# Autodesk Inventor assembly: ferris_wheel_assy1
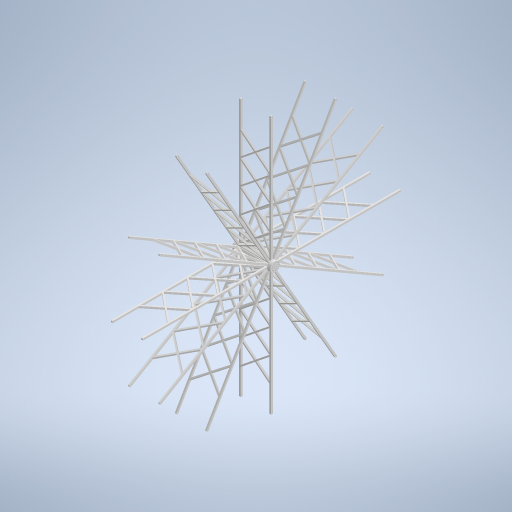
[picture p0: Inventor's stored thumbnail of the model, 512x512]
Saved by Autodesk Inventor 2023 (Build 270158000, 158)
## iProperties
Created: 2025-10-20
Part Number: ferris_wheel_assy1
Document SubType Name: Assembly
Designer: Justin Pascual
Author: Justin Pascual
## Documents named in this file (3)
- C:\Users\Justin Pascual\Documents\GitHub\amusement-park\ferris_wheel_assy1.iam
- C:\Users\Justin Pascual\Documents\GitHub\amusement-park\ferris_wheel_hub.ipt
- C:\Users\Justin Pascual\Documents\GitHub\amusement-park\ferris_wheel_main_strut.ipt
## Components (14 placed, 2 different names)
1. ferris_wheel_hub:1 — Angle:1, Mate:1, Mate:2, Mate:3, Mate:4, Mate:5, Mate:6
2. ferris_wheel_hub:2 — Mate:1, Mate:2, Mate:3
3. ferris_wheel_main_strut:1 — Mate:4, Mate:5, Angle:8
4. ferris_wheel_main_strut:2
5. ferris_wheel_main_strut:3
6. ferris_wheel_main_strut:4
7. ferris_wheel_main_strut:5
8. ferris_wheel_main_strut:6
9. ferris_wheel_main_strut:7
10. ferris_wheel_main_strut:8
11. ferris_wheel_main_strut:9
12. ferris_wheel_main_strut:10
13. ferris_wheel_main_strut:11
14. ferris_wheel_main_strut:12
## Component patterns: (12 elements, first: ferris_wheel_main_strut:1)
## Relationships (20: Mate 12, Angle 8)
- Angle:1 (0 deg): ferris_wheel_hub:1
- Mate:1: ferris_wheel_hub:1 ↔ ferris_wheel_hub:2
- Mate:2: ferris_wheel_hub:1 ↔ ferris_wheel_hub:2
- Mate:3 (63.5 mm): ferris_wheel_hub:1 ↔ ferris_wheel_hub:2
- Mate:4: ferris_wheel_hub:1 ↔ ferris_wheel_main_strut:1
- Mate:5: ferris_wheel_hub:1 ↔ ferris_wheel_main_strut:1
- Mate:6: ferris_wheel_hub:1
- Mate:7
- Angle:2 (90 deg)
- Mate:8
- Angle:3 (30 deg)
- Mate:9
- Angle:4 (60 deg)
- Mate:10
- Angle:5 (90 deg)
- Mate:11
- Angle:6 (120 deg)
- Mate:12
- Angle:7 (150 deg)
- Angle:8 (180 deg): ferris_wheel_main_strut:1
